# Autodesk Inventor assembly: 전체 조립품
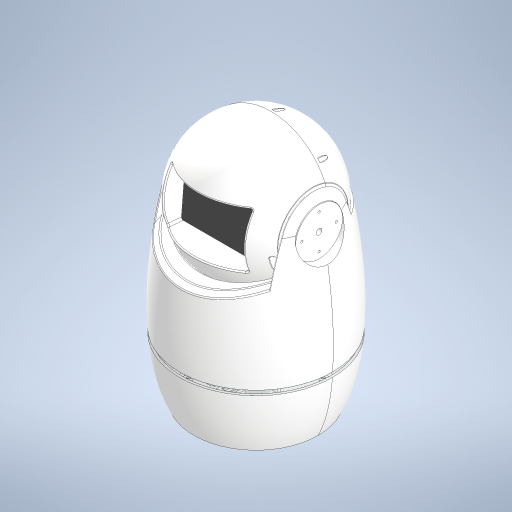
[picture p0: Inventor's stored thumbnail of the model, 512x512]
Saved by Autodesk Inventor 2023.1 (Build 271208000, 208)
## iProperties
Created: 2022-08-10
Part Number: 전체 조립품
Document SubType Name: Assembly
Designer: fly01
Author: fly01
## Documents named in this file (6)
- C:\Users\fly01\Desktop\PAI설계 2\조림품\전체 조립품.iam
- C:\Users\fly01\Desktop\PAI설계 2\조림품\머리 조립품.iam
- C:\Users\fly01\Desktop\PAI설계 2\출력품\우측 축.ipt
- C:\Users\fly01\Desktop\PAI설계 2\출력품\좌측 축.ipt
- C:\Users\fly01\Desktop\PAI설계 2\조림품\상단 조립품.iam
- C:\Users\fly01\Desktop\PAI설계 2\조림품\하단 조립품.iam
## Components (5 placed, 5 different names)
1. 머리 조립품:1 [sub-assembly] — 삽입:2
2. 우측 축:1 — 삽입:4
3. 좌측 축:1 — 삽입:3
4. 상단 조립품:1 [sub-assembly] — 삽입:1, 삽입:2, 삽입:3, 삽입:4
5. 하단 조립품:1 [sub-assembly] — 삽입:1
## Relationships (4: Insert 4)
- 삽입:1 [Insert]: 상단 조립품:1 ↔ 하단 조립품:1
- 삽입:2 [Insert] (0.5 mm): 머리 조립품:1 ↔ 상단 조립품:1
- 삽입:3 [Insert]: 좌측 축:1 ↔ 상단 조립품:1
- 삽입:4 [Insert]: 우측 축:1 ↔ 상단 조립품:1
